# Autodesk Inventor assembly: X_CarriageR_V2_0
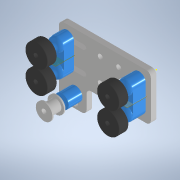
[picture p0: Inventor's stored thumbnail of the model, 180x180]
Saved by Autodesk Inventor 2021 (Build 250183000, 183)
## iProperties
Created: 2021-06-13
Part Number: X_CarriageR_V2_0
Document SubType Name: Assembly
Designer: Jorian Brusind
Author: Jorian Brusind
## Documents named in this file (8)
- C:\Users\Jorian Bruslind\Documents\GitHub\PersonalProjects\HyperRail\Inventor Files\X_CarriageR_V2_0.iam
- C:\Users\Jorian Bruslind\Documents\GitHub\PersonalProjects\HyperRail\Inventor Files\X_Carriage_Plate.ipt
- C:\Users\Jorian Bruslind\Documents\GitHub\PersonalProjects\HyperRail\Inventor Files\11mm_BearingWheel.ipt
- C:\Users\Jorian Bruslind\Documents\GitHub\PersonalProjects\HyperRail\Inventor Files\4mm_Roller_Spacer_simple.ipt
- C:\Users\Jorian Bruslind\Documents\GitHub\PersonalProjects\HyperRail\Inventor Files\4mm_Roller_Spacer_simple3mm.ipt
- C:\Users\Jorian Bruslind\Documents\GitHub\PersonalProjects\HyperRail\Inventor Files\Rollder_Spacer_Single.ipt
- C:\Users\Jorian Bruslind\Documents\GitHub\PersonalProjects\HyperRail\Inventor Files\3mm_Spacer.ipt
- C:\Users\Jorian Bruslind\Documents\GitHub\PersonalProjects\HyperRail\Inventor Files\10mm_Idle_Pulley.ipt
## Components (10 placed, 7 different names)
1. X_Carriage_Plate:1 — Mate:1, Mate:2, Mate:3, Mate:13, Mate:24, Mate:25, Mate:26, Mate:35, Mate:41, Mate:44, Mate:45
2. 11mm_BearingWheel:1 — Mate:1, Flush:2
3. 11mm_BearingWheel:2 — Flush:1, Mate:36, Mate:39
4. 11mm_BearingWheel:3 — Mate:3, Flush:1, Flush:3, Mate:47
5. 11mm_BearingWheel:4 — Mate:2, Flush:2, Flush:3
6. 4mm_Roller_Spacer_simple:1 — Mate:13, Mate:43, Mate:44, Mate:45, Mate:46, Mate:47
7. 4mm_Roller_Spacer_simple3mm:1 — Mate:24, Mate:25, Mate:26
8. Rollder_Spacer_Single:1 — Mate:35, Mate:40, Mate:41, Mate:42
9. 3mm_Spacer:1 — Mate:36, Mate:39, Mate:43, Mate:46
10. 10mm_Idle_Pulley:1 — Mate:40, Mate:42
## Relationships (21: Mate 18, Flush 3)
- Mate:1: X_Carriage_Plate:1 ↔ 11mm_BearingWheel:1
- Mate:2: X_Carriage_Plate:1 ↔ 11mm_BearingWheel:4
- Mate:3 (2.75 mm): X_Carriage_Plate:1 ↔ 11mm_BearingWheel:3
- Flush:1: 11mm_BearingWheel:2 ↔ 11mm_BearingWheel:3
- Flush:2: 11mm_BearingWheel:1 ↔ 11mm_BearingWheel:4
- Flush:3: 11mm_BearingWheel:3 ↔ 11mm_BearingWheel:4
- Mate:13: X_Carriage_Plate:1 ↔ 4mm_Roller_Spacer_simple:1
- Mate:24: X_Carriage_Plate:1 ↔ 4mm_Roller_Spacer_simple3mm:1
- Mate:25: X_Carriage_Plate:1 ↔ 4mm_Roller_Spacer_simple3mm:1
- Mate:26: X_Carriage_Plate:1 ↔ 4mm_Roller_Spacer_simple3mm:1
- Mate:35: X_Carriage_Plate:1 ↔ Rollder_Spacer_Single:1
- Mate:36: 11mm_BearingWheel:2 ↔ 3mm_Spacer:1
- Mate:39: 11mm_BearingWheel:2 ↔ 3mm_Spacer:1
- Mate:40: Rollder_Spacer_Single:1 ↔ 10mm_Idle_Pulley:1
- Mate:41: X_Carriage_Plate:1 ↔ Rollder_Spacer_Single:1
- Mate:42: Rollder_Spacer_Single:1 ↔ 10mm_Idle_Pulley:1
- Mate:43: 4mm_Roller_Spacer_simple:1 ↔ 3mm_Spacer:1
- Mate:44: X_Carriage_Plate:1 ↔ 4mm_Roller_Spacer_simple:1
- Mate:45: X_Carriage_Plate:1 ↔ 4mm_Roller_Spacer_simple:1
- Mate:46: 4mm_Roller_Spacer_simple:1 ↔ 3mm_Spacer:1
- Mate:47: 11mm_BearingWheel:3 ↔ 4mm_Roller_Spacer_simple:1
